# Autodesk Inventor assembly: Front_Frame_Fixer
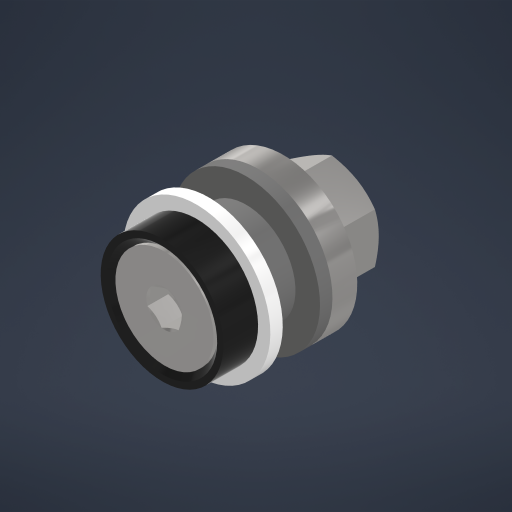
[picture p0: Inventor's stored thumbnail of the model, 512x512]
Saved by Autodesk Inventor 2024 (Build 280153000, 153)
## iProperties
Created: 2024-01-28
Part Number: Front_Frame_Fixer
Document SubType Name: Assembly
Designer: 김대겸
Author: 김대겸
## Documents named in this file (7)
- C:\Users\ASUS\Desktop\Anti_Backlash_Structure_OP\Front_Frame_Fixer.iam
- C:\Users\ASUS\Desktop\Anti_Backlash_Structure_OP\MISUMI\C-WSSA12-4-2.ipt
- C:\Users\ASUS\Desktop\Anti_Backlash_Structure_OP\Handmade tiered cover.ipt
- C:\Users\ASUS\Desktop\Anti_Backlash_Structure_OP\MISUMI\TT-0612-10.ipt
- C:\Users\ASUS\Desktop\Anti_Backlash_Structure_OP\MISUMI\80F-0603.ipt
- C:\Users\ASUS\Desktop\Anti_Backlash_Structure_OP\MISUMI\CSHCS-SUS-M4-15_214.ipt
- C:\Users\ASUS\Desktop\Anti_Backlash_Structure_OP\MISUMI\SLBNR4.ipt
## Components (6 placed, 6 different names)
1. C-WSSA12-4-2:1
2. Handmade tiered cover:1
3. TT-0612-10:1
4. 80F-0603:1
5. CSHCS-SUS-M4-15_214:1
6. SLBNR4:1
## Relationships (4: Mate 2, Insert 2)
- [Mate]: Handmade tiered cover:1 ↔ TT-0612-10:1
- [Mate]: Handmade tiered cover:1 ↔ TT-0612-10:1
- [Insert]: TT-0612-10:1 ↔ 80F-0603:1
- [Insert]: Handmade tiered cover:1 ↔ CSHCS-SUS-M4-15_214:1
